# Autodesk Inventor assembly: Gantry
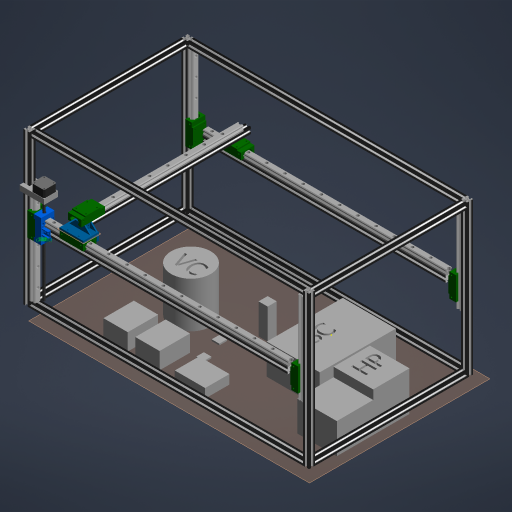
[picture p0: Inventor's stored thumbnail of the model, 512x512]
Saved by Autodesk Inventor 2024.2 (Build 282272000, 272)
## iProperties
Created: 2024-10-05
Part Number: Gantry
Document SubType Name: Assembly
Designer: jerem
Author: jerem
## Documents named in this file (24)
- C:\Users\jerem\Documents\GitHub\Perovskite-Automated-Synthesis-System\CAD\Gantry\Gantry.iam
- C:\Users\jerem\Documents\GitHub\Perovskite-Automated-Synthesis-System\CAD\Gantry\Objects\HotPlate.ipt
- C:\Users\jerem\Documents\GitHub\Perovskite-Automated-Synthesis-System\CAD\Gantry\Objects\VialCarousel.ipt
- C:\Users\jerem\Documents\GitHub\Perovskite-Automated-Synthesis-System\CAD\Gantry\Objects\TipPickup.ipt
- C:\Users\jerem\Documents\GitHub\Perovskite-Automated-Synthesis-System\CAD\Gantry\Objects\TipDropoff.ipt
- C:\Users\jerem\Documents\GitHub\Perovskite-Automated-Synthesis-System\CAD\Gantry\Objects\SpectrometerMeasurer.ipt
- C:\Users\jerem\Documents\GitHub\Perovskite-Automated-Synthesis-System\CAD\Gantry\Objects\InputStack.ipt
- C:\Users\jerem\Documents\GitHub\Perovskite-Automated-Synthesis-System\CAD\Gantry\Objects\Marker.ipt
- C:\Users\jerem\Documents\GitHub\Perovskite-Automated-Synthesis-System\CAD\Gantry\Linear Rails\HGR20 800mm.ipt
- C:\Users\jerem\Documents\GitHub\Perovskite-Automated-Synthesis-System\CAD\Gantry\Linear Rails\HGR20 300mm.ipt
- C:\Users\jerem\Documents\GitHub\Perovskite-Automated-Synthesis-System\CAD\Gantry\Extrusion\20mm Extrusion 900mm.ipt
- C:\Users\jerem\Documents\GitHub\Perovskite-Automated-Synthesis-System\CAD\Gantry\Extrusion\20mm Extrusion 500mm.ipt
- C:\Users\jerem\Documents\GitHub\Perovskite-Automated-Synthesis-System\CAD\Gantry\Extrusion\20mm Extrusion 400mm.ipt
- C:\Users\jerem\Documents\GitHub\Perovskite-Automated-Synthesis-System\CAD\Gantry\Objects\SpinCoater.ipt
- C:\Users\jerem\Documents\GitHub\Perovskite-Automated-Synthesis-System\CAD\Gantry\Linear Rails\HGH20CA Slider Block.ipt
- C:\Users\jerem\Documents\GitHub\Perovskite-Automated-Synthesis-System\CAD\Gantry\Extrusion\20mm Extrusion 800mm.ipt
- C:\Users\jerem\Documents\GitHub\Perovskite-Automated-Synthesis-System\CAD\Gantry\ZX Rail Bracket.ipt
- C:\Users\jerem\Documents\GitHub\Perovskite-Automated-Synthesis-System\CAD\Gantry\Z Stepper Holder.ipt
- C:\Users\jerem\Documents\GitHub\Perovskite-Automated-Synthesis-System\CAD\Gantry\Motors\NEMA17 Stepper Motor.ipt
- C:\Users\jerem\Documents\GitHub\Perovskite-Automated-Synthesis-System\CAD\Gantry\Threaded Rod 300mm.ipt
- C:\Users\jerem\Documents\GitHub\Perovskite-Automated-Synthesis-System\CAD\Gantry\Linear Rails\HGR20 500mm.ipt
- C:\Users\jerem\Documents\GitHub\Perovskite-Automated-Synthesis-System\CAD\Gantry\Extrusion\20mm Extrusion 550mm.ipt
- C:\Users\jerem\Documents\GitHub\Perovskite-Automated-Synthesis-System\CAD\Gantry\XY Rail Bracket.ipt
- C:\Users\jerem\Documents\GitHub\Perovskite-Automated-Synthesis-System\CAD\Gantry\Leadscrew.ipt
## Components (44 placed, 23 different names)
1. ZX Rail Bracket:1 — Mate:196, Mate:197, Mate:198, Mate:199, Mate:200, Mate:218, Mate:225, Mate:226
2. Z Stepper Holder:1 — Mate:202, Mate:203, Mate:204, Mate:228
3. NEMA17 Stepper Motor:1 — Mate:202, Mate:203, Mate:204, Mate:205, Mate:206
4. Threaded Rod 300mm:1 — Mate:205, Mate:206, Mate:218, Mate:227
5. XY Rail Bracket:1 — Mate:219, Mate:220, Mate:221, Mate:222, Mate:223, Mate:224
6. Leadscrew:1 — Mate:225, Mate:226, Mate:227
7. Marker:2 — Mate:68
8. Marker:1 — Mate:66
9. InputStack:1 — Mate:67
10. SpectrometerMeasurer:1 — Mate:62
11. TipDropoff:1 — Mate:64
12. TipPickup:1 — Mate:61
13. VialCarousel:1 — Mate:63
14. HotPlate:1 — Mate:69
15. SpinCoater:1 — Mate:65
16. 20mm Extrusion 550mm:1 — Flush:222, Mate:214, Flush:223, Mate:222, Mate:223, Mate:224
17. 20mm Extrusion 800mm:2 — Flush:216, Flush:217, Mate:195
18. 20mm Extrusion 800mm:1 — Flush:214, Mate:194, Flush:215, Mate:200
19. 20mm Extrusion 500mm:1 — Flush:163, Flush:164, Flush:166, Mate:163
20. 20mm Extrusion 400mm:1 — Flush:164, Flush:165, Flush:166, Flush:167, Mate:162, Mate:163, Flush:174, Flush:175, Mate:164, Flush:180, Flush:181, Mate:168, Flush:201, Mate:184
21. 20mm Extrusion 400mm:2 — Flush:177, Flush:178, Flush:179, Mate:167, Flush:182, Flush:183, Mate:169, Flush:184, Flush:185, Mate:172, Flush:204, Mate:189
22. 20mm Extrusion 500mm:2 — Flush:180, Flush:181, Mate:168
23. 20mm Extrusion 500mm:3 — Flush:182, Flush:183, Mate:169
24. 20mm Extrusion 500mm:4 — Mate:170, Flush:184, Flush:185, Flush:197, Flush:198, Mate:181
25. 20mm Extrusion 900mm:5 — Mate:216
26. 20mm Extrusion 900mm:6 — Mate:191
27. 20mm Extrusion 400mm:3 — Mate:228
28. 20mm Extrusion 400mm:4 — Flush:197, Flush:198, Mate:181, Mate:190, Flush:205
29. 20mm Extrusion 900mm:3 — Flush:163, Flush:165, Flush:167, Mate:162, Flush:178, Flush:179
30. 20mm Extrusion 900mm:4 — Flush:174, Flush:175, Mate:164, Flush:177, Mate:167, Mate:170, Mate:185, Mate:188
31. HGR20 500mm:1 — Mate:213, Flush:221, Flush:222, Mate:214, Flush:223
32. HGH20CA Slider Block:8 — Mate:213, Flush:221
33. HGR20 800mm:3 — Mate:192, Flush:206, Flush:214, Mate:194, Flush:215, Flush:218, Mate:199
34. HGR20 300mm:4 — Flush:199, Mate:182, Mate:216
35. HGH20CA Slider Block:1 — Flush:199, Mate:182, Flush:209, Flush:212, Mate:196, Mate:197, Mate:198
36. HGR20 300mm:6 — Flush:201, Mate:184, Mate:185, Flush:208
37. HGH20CA Slider Block:2 — Flush:210, Flush:212
38. HGR20 300mm:7 — Mate:190, Mate:191, Flush:205
39. HGH20CA Slider Block:3 — Flush:209
40. HGR20 300mm:8 — Mate:188, Flush:204, Mate:189
41. HGH20CA Slider Block:4 — Flush:210
42. HGH20CA Slider Block:5 — Mate:192, Flush:206, Flush:211, Flush:213, Mate:219, Mate:220, Mate:221
43. HGR20 800mm:4 — Flush:208, Flush:216, Flush:217, Mate:195, Flush:218
44. HGH20CA Slider Block:6 — Flush:211, Flush:213
## Relationships (109: Mate 60, Flush 49)
- Flush:140 (-50 mm)
- Mate:61: TipPickup:1
- Mate:62: SpectrometerMeasurer:1
- Mate:63: VialCarousel:1
- Mate:64: TipDropoff:1
- Mate:65: SpinCoater:1
- Mate:66: Marker:1
- Mate:67: InputStack:1
- Mate:68: Marker:2
- Mate:69: HotPlate:1
- Flush:163: 20mm Extrusion 500mm:1 ↔ 20mm Extrusion 900mm:3
- Flush:164: 20mm Extrusion 500mm:1 ↔ 20mm Extrusion 400mm:1
- Flush:165: 20mm Extrusion 400mm:1 ↔ 20mm Extrusion 900mm:3
- Flush:166: 20mm Extrusion 500mm:1 ↔ 20mm Extrusion 400mm:1
- Flush:167: 20mm Extrusion 400mm:1 ↔ 20mm Extrusion 900mm:3
- Mate:162: 20mm Extrusion 400mm:1 ↔ 20mm Extrusion 900mm:3
- Mate:163: 20mm Extrusion 500mm:1 ↔ 20mm Extrusion 400mm:1
- Flush:174: 20mm Extrusion 400mm:1 ↔ 20mm Extrusion 900mm:4
- Flush:175: 20mm Extrusion 400mm:1 ↔ 20mm Extrusion 900mm:4
- Mate:164: 20mm Extrusion 400mm:1 ↔ 20mm Extrusion 900mm:4
- Flush:177: 20mm Extrusion 400mm:2 ↔ 20mm Extrusion 900mm:4
- Flush:178: 20mm Extrusion 400mm:2 ↔ 20mm Extrusion 900mm:3
- Flush:179: 20mm Extrusion 400mm:2 ↔ 20mm Extrusion 900mm:3
- Mate:167: 20mm Extrusion 400mm:2 ↔ 20mm Extrusion 900mm:4
- Flush:180: 20mm Extrusion 400mm:1 ↔ 20mm Extrusion 500mm:2
- Flush:181: 20mm Extrusion 400mm:1 ↔ 20mm Extrusion 500mm:2
- Mate:168: 20mm Extrusion 400mm:1 ↔ 20mm Extrusion 500mm:2
- Flush:182: 20mm Extrusion 400mm:2 ↔ 20mm Extrusion 500mm:3
- Flush:183: 20mm Extrusion 400mm:2 ↔ 20mm Extrusion 500mm:3
- Mate:169: 20mm Extrusion 400mm:2 ↔ 20mm Extrusion 500mm:3
- Mate:170: 20mm Extrusion 500mm:4 ↔ 20mm Extrusion 900mm:4
- Flush:184: 20mm Extrusion 400mm:2 ↔ 20mm Extrusion 500mm:4
- Flush:185: 20mm Extrusion 400mm:2 ↔ 20mm Extrusion 500mm:4
- Mate:172: 20mm Extrusion 400mm:2
- [Flush]: HGR20 800mm:3 ↔ HGR20 300mm:4
- [Flush]: 20mm Extrusion 900mm:5 ↔ 20mm Extrusion 400mm:3
- [Flush]: 20mm Extrusion 900mm:5 ↔ 20mm Extrusion 400mm:3
- [Mate]: 20mm Extrusion 900mm:5 ↔ 20mm Extrusion 400mm:3
- [Flush]: 20mm Extrusion 900mm:6 ↔ 20mm Extrusion 400mm:3
- [Mate]: 20mm Extrusion 900mm:6 ↔ 20mm Extrusion 400mm:3
- [Mate]: 20mm Extrusion 400mm:3 ↔ HGR20 300mm:4
- [Flush]: 20mm Extrusion 400mm:3 ↔ HGR20 300mm:4
- [Flush]: 20mm Extrusion 900mm:5 ↔ 20mm Extrusion 400mm:4
- [Flush]: 20mm Extrusion 900mm:5 ↔ 20mm Extrusion 400mm:4
- [Mate]: 20mm Extrusion 900mm:6 ↔ 20mm Extrusion 400mm:4
- Flush:197: 20mm Extrusion 500mm:4 ↔ 20mm Extrusion 400mm:4
- Flush:198: 20mm Extrusion 500mm:4 ↔ 20mm Extrusion 400mm:4
- Mate:181: 20mm Extrusion 500mm:4 ↔ 20mm Extrusion 400mm:4
- Flush:199 (-4.6 mm): HGR20 300mm:4 ↔ HGH20CA Slider Block:1
- Mate:182: HGR20 300mm:4 ↔ HGH20CA Slider Block:1
- [Flush] (-4.6 mm): HGR20 300mm:6 ↔ HGH20CA Slider Block:2
- [Mate]: HGR20 300mm:6 ↔ HGH20CA Slider Block:2
- Flush:201: 20mm Extrusion 400mm:1 ↔ HGR20 300mm:6
- Mate:184: 20mm Extrusion 400mm:1 ↔ HGR20 300mm:6
- Mate:185: 20mm Extrusion 900mm:4 ↔ HGR20 300mm:6
- [Flush] (-4.6 mm): HGR20 300mm:7 ↔ HGH20CA Slider Block:3
- [Mate]: HGR20 300mm:7 ↔ HGH20CA Slider Block:3
- [Flush] (-4.6 mm): HGR20 300mm:8 ↔ HGH20CA Slider Block:4
- [Mate]: HGR20 300mm:8 ↔ HGH20CA Slider Block:4
- Mate:188: 20mm Extrusion 900mm:4 ↔ HGR20 300mm:8
- Flush:204: 20mm Extrusion 400mm:2 ↔ HGR20 300mm:8
- Mate:189: 20mm Extrusion 400mm:2 ↔ HGR20 300mm:8
- Mate:190: 20mm Extrusion 400mm:4 ↔ HGR20 300mm:7
- Mate:191: 20mm Extrusion 900mm:6 ↔ HGR20 300mm:7
- Flush:205: 20mm Extrusion 400mm:4 ↔ HGR20 300mm:7
- Mate:192: HGR20 800mm:3 ↔ HGH20CA Slider Block:5
- Flush:206 (4.6 mm): HGR20 800mm:3 ↔ HGH20CA Slider Block:5
- [Mate]: HGR20 800mm:4 ↔ HGH20CA Slider Block:6
- [Flush] (4.6 mm): HGR20 800mm:4 ↔ HGH20CA Slider Block:6
- Flush:208: HGR20 300mm:6 ↔ HGR20 800mm:4
- Flush:209: HGH20CA Slider Block:1 ↔ HGH20CA Slider Block:3
- Flush:210: HGH20CA Slider Block:2 ↔ HGH20CA Slider Block:4
- Flush:211: HGH20CA Slider Block:5 ↔ HGH20CA Slider Block:6
- Flush:212: HGH20CA Slider Block:1 ↔ HGH20CA Slider Block:2
- Flush:213: HGH20CA Slider Block:5 ↔ HGH20CA Slider Block:6
- Flush:214: 20mm Extrusion 800mm:1 ↔ HGR20 800mm:3
- Mate:194: 20mm Extrusion 800mm:1 ↔ HGR20 800mm:3
- Flush:215: 20mm Extrusion 800mm:1 ↔ HGR20 800mm:3
- Flush:216: 20mm Extrusion 800mm:2 ↔ HGR20 800mm:4
- Flush:217: 20mm Extrusion 800mm:2 ↔ HGR20 800mm:4
- Mate:195: 20mm Extrusion 800mm:2 ↔ HGR20 800mm:4
- Flush:218: HGR20 800mm:3 ↔ HGR20 800mm:4
- Mate:196: ZX Rail Bracket:1 ↔ HGH20CA Slider Block:1
- Mate:197: ZX Rail Bracket:1 ↔ HGH20CA Slider Block:1
- Mate:198: ZX Rail Bracket:1 ↔ HGH20CA Slider Block:1
- Mate:199: ZX Rail Bracket:1 ↔ HGR20 800mm:3
- Mate:200: ZX Rail Bracket:1 ↔ 20mm Extrusion 800mm:1
- Mate:202: Z Stepper Holder:1 ↔ NEMA17 Stepper Motor:1
- Mate:203: Z Stepper Holder:1 ↔ NEMA17 Stepper Motor:1
- Mate:204: Z Stepper Holder:1 ↔ NEMA17 Stepper Motor:1
- Mate:205: NEMA17 Stepper Motor:1 ↔ Threaded Rod 300mm:1
- Mate:206: NEMA17 Stepper Motor:1 ↔ Threaded Rod 300mm:1
- Mate:213: HGR20 500mm:1 ↔ HGH20CA Slider Block:8
- Flush:221 (4.6 mm): HGR20 500mm:1 ↔ HGH20CA Slider Block:8
- Flush:222: 20mm Extrusion 550mm:1 ↔ HGR20 500mm:1
- Mate:214: 20mm Extrusion 550mm:1 ↔ HGR20 500mm:1
- Mate:216: 20mm Extrusion 900mm:5 ↔ HGR20 300mm:4
- Mate:218: ZX Rail Bracket:1 ↔ Threaded Rod 300mm:1
- Flush:223 (25 mm): 20mm Extrusion 550mm:1 ↔ HGR20 500mm:1
- Mate:219: XY Rail Bracket:1 ↔ HGH20CA Slider Block:5
- Mate:220: XY Rail Bracket:1 ↔ HGH20CA Slider Block:5
- Mate:221: XY Rail Bracket:1 ↔ HGH20CA Slider Block:5
- Mate:222: XY Rail Bracket:1 ↔ 20mm Extrusion 550mm:1
- Mate:223: XY Rail Bracket:1 ↔ 20mm Extrusion 550mm:1
- Mate:224: XY Rail Bracket:1 ↔ 20mm Extrusion 550mm:1
- Mate:225: ZX Rail Bracket:1 ↔ Leadscrew:1
- Mate:226: ZX Rail Bracket:1 ↔ Leadscrew:1
- Mate:227: Threaded Rod 300mm:1 ↔ Leadscrew:1
- Mate:228: Z Stepper Holder:1 ↔ 20mm Extrusion 400mm:3
## Named parameters: d281_d262 = 0 mm, d282_d263 = 0 mm, d285_d266 = 0 mm, d286_d267 = 0 mm, d287_d268 = 0 mm, d288_d248 = 0 mm, d289_d250 = 0 mm, d290_d251 = 0 mm, d292_d260 = 0 mm, d293_d261 = 0 mm, d296_d237 = 0 mm, d304_d302 = -4.6 mm, d305_d303 = 0 mm, d309_d302 = -4.6 mm, d310_d303 = 0 mm, d311_d304_d302 = -4.6 mm, d312_d305_d303 = 0 mm, d321_d319 = 0 mm, d322_d320 = 4.6 mm
